# Autodesk Inventor assembly: 200-20-ROCKER-CONNECTOR-ASM-01
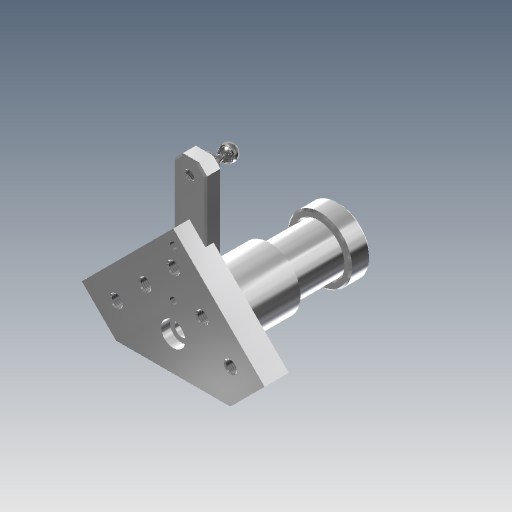
[picture p0: Inventor's stored thumbnail of the model, 512x512]
Saved by Autodesk Inventor 2018.2 (Build 222227000, 227)
## iProperties
Manager: feesmrt
Company: FRANC0R
Created: 2017-11-01
Part Number: 200-20-ROCKER-CONNECTOR-ASM-01
Material: Generisch
Document SubType Name: Assembly
Designer: feesmrt
Project: Rescue Robot
Cost Center: -
Description: Rocker Bearing Connector
Engineer: feesmrt
Authority: feesmrt
Stock Number: 200-20-ROCKER-CONNECTOR-ASM-01
Mass: 342.249 g
Surface Area: 374.371 cm^2
Volume: 115.439 cm^3
Density: 2.96477 g/cm^3
Author: feesmrt
Title: Rocker Bearing Connector
Subject: Rescue Robot
Revision Number: 1
## Documents named in this file (6)
- D:\Programmierung\FRANC0R\CAD\02-Rocker-Bogie-Robot\200-ROCKER-BOGIE\200-20-ROCKER-CONNECTOR\200-20-ROCKER-CONNECTOR-ASM-01.iam
- D:\Programmierung\FRANC0R\CAD\02-Rocker-Bogie-Robot\200-ROCKER-BOGIE\200-20-ROCKER-CONNECTOR\200-20-ROCKER-CONNECTOR-01.ipt
- D:\Programmierung\FRANC0R\CAD\02-Rocker-Bogie-Robot\200-ROCKER-BOGIE\200-20-ROCKER-CONNECTOR\200-20-ROCKER-CONNECTOR-02.ipt
- D:\Programmierung\FRANC0R\CAD\02-Rocker-Bogie-Robot\900-COMPONENTS\900-40-SCREWS\900-40-SCREWS-ISO10642_M6x16.ipt
- D:\Programmierung\FRANC0R\CAD\02-Rocker-Bogie-Robot\200-ROCKER-BOGIE\200-20-ROCKER-CONNECTOR\200-20-ROCKER-CONNECTOR-04.ipt
- D:\Programmierung\FRANC0R\CAD\02-Rocker-Bogie-Robot\200-ROCKER-BOGIE\200-60-DIFFERENTIAL\200-60-DIFFERENTIAL-BAR-01.iam
## Components (5 placed, 5 different names)
1. 200-20-ROCKER-CONNECTOR-01:1 — Passend:1, Passend:2, Passend:29, Passend:30, Passend:31
2. 200-20-ROCKER-CONNECTOR-02:1 — Passend:1, Passend:2, Passend:4, Fluchtend:1
3. 900-40-SCREWS-ISO10642_M6x16:1 — Passend:4, Fluchtend:1
4. 200-20-ROCKER-CONNECTOR-04:1 — Passend:29, Passend:30, Passend:31, Passend:32, Passend:33, Passend:34
5. 200-60-DIFFERENTIAL-BAR-01:1 [sub-assembly] — Passend:32, Passend:33, Passend:34
## Relationships (10: Mate 9, Flush 1)
- Passend:1 [Mate]: 200-20-ROCKER-CONNECTOR-01:1 ↔ 200-20-ROCKER-CONNECTOR-02:1
- Passend:2 [Mate]: 200-20-ROCKER-CONNECTOR-01:1 ↔ 200-20-ROCKER-CONNECTOR-02:1
- Passend:4 [Mate]: 200-20-ROCKER-CONNECTOR-02:1 ↔ 900-40-SCREWS-ISO10642_M6x16:1
- Fluchtend:1 [Flush]: 200-20-ROCKER-CONNECTOR-02:1 ↔ 900-40-SCREWS-ISO10642_M6x16:1
- Passend:29 [Mate]: 200-20-ROCKER-CONNECTOR-01:1 ↔ 200-20-ROCKER-CONNECTOR-04:1
- Passend:30 [Mate]: 200-20-ROCKER-CONNECTOR-01:1 ↔ 200-20-ROCKER-CONNECTOR-04:1
- Passend:31 [Mate]: 200-20-ROCKER-CONNECTOR-01:1 ↔ 200-20-ROCKER-CONNECTOR-04:1
- Passend:32 [Mate]: 200-20-ROCKER-CONNECTOR-04:1 ↔ 200-60-DIFFERENTIAL-BAR-01:1
- Passend:33 [Mate]: 200-20-ROCKER-CONNECTOR-04:1 ↔ 200-60-DIFFERENTIAL-BAR-01:1
- Passend:34 [Mate]: 200-20-ROCKER-CONNECTOR-04:1 ↔ 200-60-DIFFERENTIAL-BAR-01:1
